# Autodesk Inventor assembly: GPS-TRACKER_V2
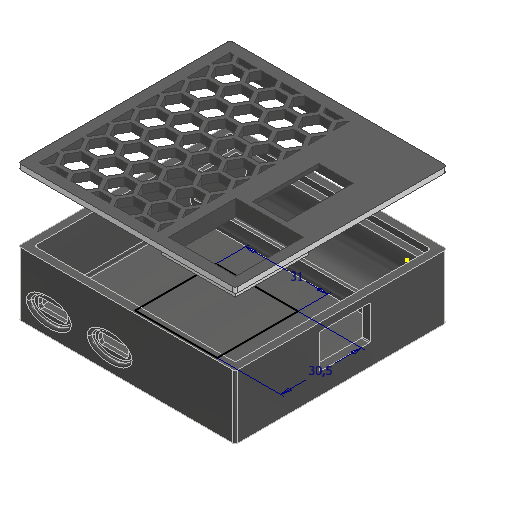
[picture p0: Inventor's stored thumbnail of the model, 512x512]
Saved by Autodesk Inventor 2026.1 (Build 301233020, 233B)
## iProperties
Created: 2026-01-15
Part Number: GPS-TRACKER_V2
Document SubType Name: Assembly
Designer: Paweł
Author: Paweł
## Documents named in this file (3)
- C:\Users\Paweł\OneDrive - Politechnika Warszawska\Dokumenty\GPS-Tracker\Models_Inventor\GPS-TRACKER_V2.iam
- C:\Users\Paweł\OneDrive - Politechnika Warszawska\Dokumenty\GPS-Tracker\Models_Inventor\pudelko_v2.ipt
- C:\Users\Paweł\OneDrive - Politechnika Warszawska\Dokumenty\GPS-Tracker\Models_Inventor\FINALPOKRYWKAV2.ipt
## Components (2 placed, 2 different names)
1. pudelko_v2:1 — Mate:1, Mate:2
2. FINALPOKRYWKAV2:1 — Mate:1, Mate:2
## Relationships (2: Mate 2)
- Mate:1: pudelko_v2:1 ↔ FINALPOKRYWKAV2:1
- Mate:2: pudelko_v2:1 ↔ FINALPOKRYWKAV2:1
